# Autodesk Inventor assembly: Фильтр D1000
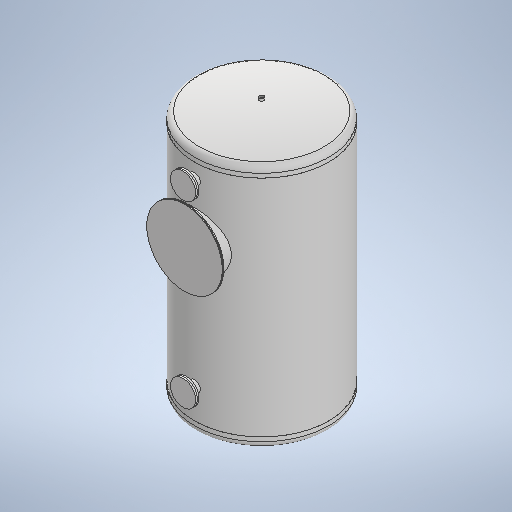
[picture p0: Inventor's stored thumbnail of the model, 512x512]
Saved by Autodesk Inventor 2025 (Build 290162010, 162A)
## iProperties
Created: 2025-02-12
Part Number: Фильтр D1000
Document SubType Name: Assembly
Designer: pokla
Author: pokla
## Documents named in this file (11)
- C:\Users\pokla\Desktop\Работа Акватроник\Фильтры напорные\D1000\Фильтр D1000.iam
- C:\Users\pokla\Desktop\Работа Акватроник\Фильтры напорные\D1000\Стенка фильтра D1000.ipt
- C:\Users\pokla\Desktop\Работа Акватроник\Фильтры напорные\D1000\Размеры D1000.ipt
- C:\Users\pokla\Desktop\Работа Акватроник\Фильтры напорные\D1000\Ревиз. окно фильтра D1000.ipt
- C:\Users\pokla\Desktop\Работа Акватроник\Фильтры напорные\D1000\Кольцо заглушки ревиз. окна фильтра D1000.ipt
- C:\Users\pokla\Desktop\Работа Акватроник\Фильтры напорные\D1000\Заглушка ревиз. окна фильтра D1000.ipt
- C:\Users\pokla\Desktop\Работа Акватроник\Фильтры напорные\D1000\Труба подключения фильтра D1000.ipt
- C:\Users\pokla\Desktop\Работа Акватроник\Фильтры напорные\D1000\Фланец трубы подключения фильтра D1000.ipt
- C:\Users\pokla\Desktop\Работа Акватроник\Фильтры напорные\D1000\Заглушка фланца трубы подключения фильтра D1000.ipt
- C:\Users\pokla\Desktop\Работа Акватроник\Фильтры напорные\D1000\Сферическое дно D1000.ipt
- C:\Users\pokla\Desktop\Работа Акватроник\Фильтры напорные\D1000\Штуцер фильтра D1000.ipt
## Components (18 placed, 10 different names)
1. Размеры D1000:1
2. Стенка фильтра D1000:1 — Mate:1, Flush:1, Rigid:7, Rigid:11, Rigid:12, Rigid:13
3. Ревиз. окно фильтра D1000:1 — Mate:1, Flush:1, Flush:2, Rigid:2
4. Кольцо заглушки ревиз. окна фильтра D1000:1 — Rigid:1, Rigid:2, Rigid:3
5. Кольцо заглушки ревиз. окна фильтра D1000:2 — Rigid:1
6. Заглушка ревиз. окна фильтра D1000:1 — Rigid:3
7. Труба подключения фильтра D1000:1 — Rigid:4, Rigid:5, Rigid:7
8. Фланец трубы подключения фильтра D1000:1 — Rigid:4, Rigid:6
9. Фланец трубы подключения фильтра D1000:2 — Rigid:5
10. Заглушка фланца трубы подключения фильтра D1000:1 — Rigid:6
11. Труба подключения фильтра D1000:2 — Rigid:11
12. Фланец трубы подключения фильтра D1000:3
13. Заглушка фланца трубы подключения фильтра D1000:2
14. Фланец трубы подключения фильтра D1000:4
15. Сферическое дно D1000:1 — Rigid:12, Rigid:15
16. Сферическое дно D1000:2 — Rigid:13, Rigid:14
17. Штуцер фильтра D1000:1 — Rigid:14
18. Штуцер фильтра D1000:2 — Rigid:15
## Relationships (18: WeldJoint 15, Flush 2, Mate 1)
- Mate:1: Стенка фильтра D1000:1 ↔ Ревиз. окно фильтра D1000:1
- Flush:1 (495 mm): Стенка фильтра D1000:1 ↔ Ревиз. окно фильтра D1000:1
- Flush:2: Ревиз. окно фильтра D1000:1
- Rigid:1 [WeldJoint]: Кольцо заглушки ревиз. окна фильтра D1000:1 ↔ Кольцо заглушки ревиз. окна фильтра D1000:2
- Rigid:2 [WeldJoint]: Ревиз. окно фильтра D1000:1 ↔ Кольцо заглушки ревиз. окна фильтра D1000:1
- Rigid:3 [WeldJoint]: Кольцо заглушки ревиз. окна фильтра D1000:1 ↔ Заглушка ревиз. окна фильтра D1000:1
- Rigid:4 [WeldJoint]: Труба подключения фильтра D1000:1 ↔ Фланец трубы подключения фильтра D1000:1
- Rigid:5 [WeldJoint]: Труба подключения фильтра D1000:1 ↔ Фланец трубы подключения фильтра D1000:2
- Rigid:6 [WeldJoint]: Фланец трубы подключения фильтра D1000:1 ↔ Заглушка фланца трубы подключения фильтра D1000:1
- Rigid:7 [WeldJoint] (97 mm): Стенка фильтра D1000:1 ↔ Труба подключения фильтра D1000:1
- [WeldJoint]: Труба подключения фильтра D1000:2 ↔ Фланец трубы подключения фильтра D1000:3
- [WeldJoint]: Труба подключения фильтра D1000:2 ↔ Фланец трубы подключения фильтра D1000:4
- [WeldJoint]: Фланец трубы подключения фильтра D1000:3 ↔ Заглушка фланца трубы подключения фильтра D1000:2
- Rigid:11 [WeldJoint] (97 mm): Стенка фильтра D1000:1 ↔ Труба подключения фильтра D1000:2
- Rigid:12 [WeldJoint]: Стенка фильтра D1000:1 ↔ Сферическое дно D1000:1
- Rigid:13 [WeldJoint]: Стенка фильтра D1000:1 ↔ Сферическое дно D1000:2
- Rigid:14 [WeldJoint]: Сферическое дно D1000:2 ↔ Штуцер фильтра D1000:1
- Rigid:15 [WeldJoint]: Сферическое дно D1000:1 ↔ Штуцер фильтра D1000:2
## Named parameters: d13_d7 = 0 mm, d14_d8 = 0 mm, d15_d11 = 0 mm
